# Autodesk Inventor assembly: motor
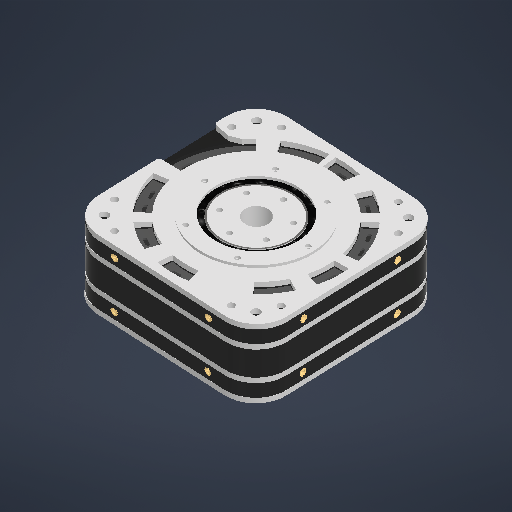
[picture p0: Inventor's stored thumbnail of the model, 512x512]
Saved by Autodesk Inventor 2026.1 (Build 301233000, 233)
## iProperties
Created: 2025-03-05
Part Number: motor
Document SubType Name: Assembly
Designer: aaron
Author: aaron
## Documents named in this file (11)
- D:\work\loopandpixel\openworkoutsystem\cad\v5\motor.iam
- D:\work\loopandpixel\openworkoutsystem\cad\v5\RI115-PH\RI115-PH.iam
- D:\work\loopandpixel\openworkoutsystem\cad\v5\bearings\bearing_58x45x7.ipt
- D:\work\loopandpixel\openworkoutsystem\cad\v5\rotor_hub_drive_side.ipt
- D:\work\loopandpixel\openworkoutsystem\cad\v5\stator_mount_01_alu.ipt
- D:\work\loopandpixel\openworkoutsystem\cad\v5\stator_center_00_alu.ipt
- D:\work\loopandpixel\openworkoutsystem\cad\v5\stator_center_01_p.ipt
- D:\work\loopandpixel\openworkoutsystem\cad\v5\stator_mount_ret.ipt
- D:\work\loopandpixel\openworkoutsystem\cad\v5\stator_center_00_p.ipt
- D:\work\loopandpixel\openworkoutsystem\cad\v5\stator_center_01_back_p.ipt
- D:\work\loopandpixel\openworkoutsystem\cad\v5\ruthex_RX-M3x5_7\ruthex_RX-M3x5_7\ruthex_RX-M3x5_7.iam
## Components (30 placed, 10 different names)
1. RI115-PH:1 [sub-assembly] — Insert:9, Insert:10, Mate:23, Mate:26, Mate:27, Mate:28, Mate:31, Insert:22
2. bearing_58x45x7:1 — Insert:11, Mate:16
3. rotor_hub_drive_side:1 — Insert:10, Insert:12
4. stator_mount_01_alu:1 — Mate:18, Flush:4
5. bearing_58x45x7:2 — Insert:12, Mate:18, Insert:20
6. rotor_hub_drive_side:2 — Insert:9, Insert:11, Flush:1
7. stator_mount_01_alu:2 — Mate:16, Insert:19, Flush:1, Flush:3
8. stator_center_01_p:1 — Mate:23, Insert:16, Insert:24, Insert:26, Insert:27, Insert:29, Insert:32, Insert:34, Insert:36, Insert:38
9. stator_center_00_alu:1 — Mate:26, Insert:13, Insert:21
10. stator_center_00_alu:2 — Mate:27, Insert:15, Insert:16, Flush:3
11. stator_center_00_p:1 — Mate:28, Insert:13, Insert:15
12. stator_mount_ret:2 — Insert:19
13. stator_mount_ret:3 — Insert:20
14. stator_center_01_back_p:1 — Mate:31, Insert:21, Insert:22, Insert:23, Insert:25, Insert:28, Insert:30, Insert:31, Insert:33, Insert:35, Insert:37, Flush:4
15. ruthex_RX-M3x5_7:1 [sub-assembly] — Insert:23
16. ruthex_RX-M3x5_7:2 [sub-assembly] — Insert:30
17. ruthex_RX-M3x5_7:3 [sub-assembly] — Insert:31
18. ruthex_RX-M3x5_7:4 [sub-assembly] — Insert:32
19. ruthex_RX-M3x5_7:5 [sub-assembly] — Insert:33
20. ruthex_RX-M3x5_7:6 [sub-assembly] — Insert:29
21. ruthex_RX-M3x5_7:7 [sub-assembly] — Insert:27
22. ruthex_RX-M3x5_7:8 [sub-assembly] — Insert:28
23. ruthex_RX-M3x5_7:9 [sub-assembly] — Insert:26
24. ruthex_RX-M3x5_7:10 [sub-assembly] — Insert:25
25. ruthex_RX-M3x5_7:11 [sub-assembly] — Insert:24
26. ruthex_RX-M3x5_7:12 [sub-assembly] — Insert:34
27. ruthex_RX-M3x5_7:13 [sub-assembly] — Insert:38
28. ruthex_RX-M3x5_7:14 [sub-assembly] — Insert:37
29. ruthex_RX-M3x5_7:15 [sub-assembly] — Insert:36
30. ruthex_RX-M3x5_7:16 [sub-assembly] — Insert:35
## Relationships (37: Insert 27, Mate 7, Flush 3)
- Insert:9: RI115-PH:1 ↔ rotor_hub_drive_side:2
- Insert:10: RI115-PH:1 ↔ rotor_hub_drive_side:1
- Insert:11: bearing_58x45x7:1 ↔ rotor_hub_drive_side:2
- Insert:12: rotor_hub_drive_side:1 ↔ bearing_58x45x7:2
- Mate:16: bearing_58x45x7:1 ↔ stator_mount_01_alu:2
- Mate:18: stator_mount_01_alu:1 ↔ bearing_58x45x7:2
- Mate:23: RI115-PH:1 ↔ stator_center_01_p:1
- Mate:26: RI115-PH:1 ↔ stator_center_00_alu:1
- Mate:27: RI115-PH:1 ↔ stator_center_00_alu:2
- Mate:28: RI115-PH:1 ↔ stator_center_00_p:1
- Insert:13: stator_center_00_alu:1 ↔ stator_center_00_p:1
- Insert:15: stator_center_00_alu:2 ↔ stator_center_00_p:1
- Insert:16: stator_center_01_p:1 ↔ stator_center_00_alu:2
- Insert:19: stator_mount_01_alu:2 ↔ stator_mount_ret:2
- Flush:1: rotor_hub_drive_side:2 ↔ stator_mount_01_alu:2
- Insert:20: bearing_58x45x7:2 ↔ stator_mount_ret:3
- Flush:3: stator_mount_01_alu:2 ↔ stator_center_00_alu:2
- Mate:31: RI115-PH:1 ↔ stator_center_01_back_p:1
- Insert:21: stator_center_00_alu:1 ↔ stator_center_01_back_p:1
- Insert:22: RI115-PH:1 ↔ stator_center_01_back_p:1
- Insert:23: stator_center_01_back_p:1 ↔ ruthex_RX-M3x5_7:1
- Insert:24: stator_center_01_p:1 ↔ ruthex_RX-M3x5_7:11
- Insert:25: stator_center_01_back_p:1 ↔ ruthex_RX-M3x5_7:10
- Insert:26: stator_center_01_p:1 ↔ ruthex_RX-M3x5_7:9
- Insert:27: stator_center_01_p:1 ↔ ruthex_RX-M3x5_7:7
- Insert:28: stator_center_01_back_p:1 ↔ ruthex_RX-M3x5_7:8
- Insert:29: stator_center_01_p:1 ↔ ruthex_RX-M3x5_7:6
- Insert:30: stator_center_01_back_p:1 ↔ ruthex_RX-M3x5_7:2
- Insert:31: stator_center_01_back_p:1 ↔ ruthex_RX-M3x5_7:3
- Insert:32: stator_center_01_p:1 ↔ ruthex_RX-M3x5_7:4
- Insert:33: stator_center_01_back_p:1 ↔ ruthex_RX-M3x5_7:5
- Insert:34: stator_center_01_p:1 ↔ ruthex_RX-M3x5_7:12
- Insert:35: stator_center_01_back_p:1 ↔ ruthex_RX-M3x5_7:16
- Insert:36: stator_center_01_p:1 ↔ ruthex_RX-M3x5_7:15
- Insert:37: stator_center_01_back_p:1 ↔ ruthex_RX-M3x5_7:14
- Insert:38: stator_center_01_p:1 ↔ ruthex_RX-M3x5_7:13
- Flush:4: stator_mount_01_alu:1 ↔ stator_center_01_back_p:1
